# Autodesk Inventor assembly: V-Belt transmission
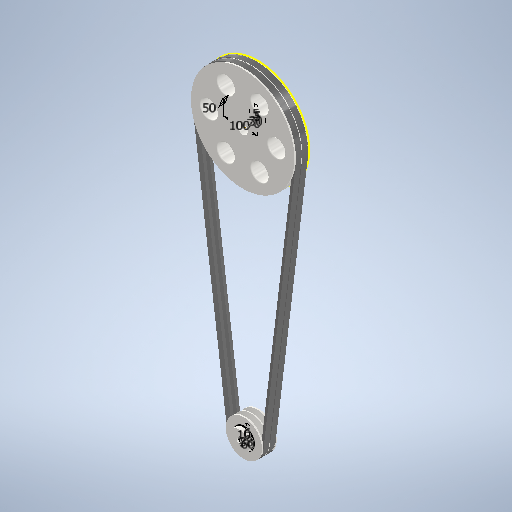
[picture p0: Inventor's stored thumbnail of the model, 512x512]
Saved by Autodesk Inventor 2025 (Build 290162000, 162)
## iProperties
ClientObjectVersion: 1
Created: 2025-05-25
Part Number: V-Belt transmission
Document SubType Name: Assembly
Designer: Abdullah
Author: Abdullah
## Documents named in this file (4)
- D:\A-Engineering\SENIOR1_MCT_SEC_TERM\MDP494s- Advanced Manufacturing Technology & Prototyping\poject\New folder (2)\V-Belt transmission.iam
- D:\A-Engineering\SENIOR1_MCT_SEC_TERM\MDP494s- Advanced Manufacturing Technology & Prototyping\poject\New folder (2)\V-Belt.ipt
- D:\A-Engineering\SENIOR1_MCT_SEC_TERM\MDP494s- Advanced Manufacturing Technology & Prototyping\poject\New folder (2)\Grooved Pulley1.ipt
- D:\A-Engineering\SENIOR1_MCT_SEC_TERM\MDP494s- Advanced Manufacturing Technology & Prototyping\poject\New folder (2)\Grooved Pulley2.ipt
## Components (4 placed, 3 different names)
1. Grooved Pulley1:1 — Flush:1, Mate:1, Rotation:1
2. Grooved Pulley2:1 — Flush:2, Mate:2, Rotation:1
3. V-Belt:1 — Flush:1, Mate:1, Flush:2, Mate:2
4. V-Belt:2
## Component patterns: (2 elements, first: V-Belt:1)
## Relationships (5: Flush 2, Mate 2, RelateRotation 1)
- Flush:1: Grooved Pulley1:1 ↔ V-Belt:1
- Mate:1: Grooved Pulley1:1 ↔ V-Belt:1
- Flush:2: Grooved Pulley2:1 ↔ V-Belt:1
- Mate:2: Grooved Pulley2:1 ↔ V-Belt:1
- Rotation:1 [RelateRotation] (3 ul): Grooved Pulley1:1 ↔ Grooved Pulley2:1
